# Autodesk Inventor assembly: Escaner3D
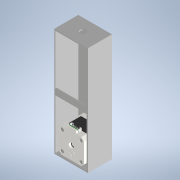
[picture p0: Inventor's stored thumbnail of the model, 180x180]
Saved by Autodesk Inventor 2020 (Build 240168000, 168)
## iProperties
Created: 2023-03-22
Part Number: Escaner3D
Document SubType Name: Assembly
Designer: semon
Author: semon
## Documents named in this file (3)
- C:\Users\semon\OneDrive - Universidad Nacional de Colombia\GitHub\semontoya_TallerV\Proyecto\Diseño\Escaner3D.iam
- C:\Users\semon\OneDrive - Universidad Nacional de Colombia\GitHub\semontoya_TallerV\Proyecto\Diseño\Soporte_base.ipt
- C:\Users\semon\OneDrive - Universidad Nacional de Colombia\GitHub\semontoya_TallerV\Proyecto\Diseño\Nema 17 Motor a Pasos 17HS4401.ipt
## Components (2 placed, 2 different names)
1. Soporte_base:1 — Mate:1, Mate:2, Mate:3
2. Nema 17 Motor a Pasos 17HS4401:1 — Mate:1, Mate:2, Mate:3
## Relationships (3: Mate 3)
- Mate:1: Soporte_base:1 ↔ Nema 17 Motor a Pasos 17HS4401:1
- Mate:2: Soporte_base:1 ↔ Nema 17 Motor a Pasos 17HS4401:1
- Mate:3: Soporte_base:1 ↔ Nema 17 Motor a Pasos 17HS4401:1
